# Autodesk Inventor assembly: Full_Model
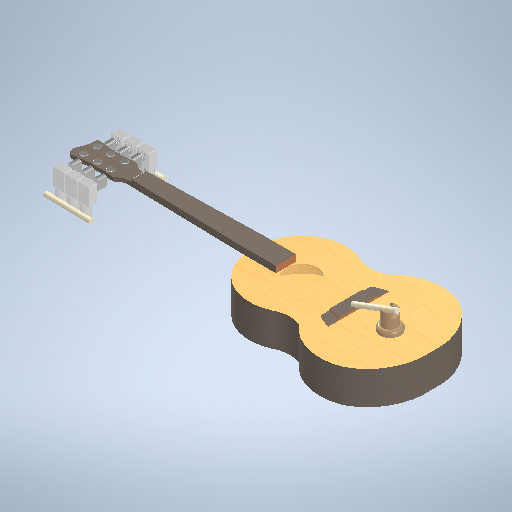
[picture p0: Inventor's stored thumbnail of the model, 512x512]
Saved by Autodesk Inventor 2025.2 (Build 292293000, 293)
## iProperties
Created: 2025-04-14
Part Number: Full_Model
Document SubType Name: Assembly
Designer: 3lin2
Author: 3lin2
## Documents named in this file (7)
- C:\Users\3lin2\OneDrive - University of Illinois - Urbana\Documents\UIUC\ECE 445\Automatic-Guitar-Tuner Github\3D_print\Full_Model.iam
- C:\Users\3lin2\OneDrive - University of Illinois - Urbana\Documents\UIUC\ECE 445\Automatic-Guitar-Tuner Github\3D_print\half_inch_dowel_5inch.ipt
- C:\Users\3lin2\OneDrive - University of Illinois - Urbana\Documents\UIUC\ECE 445\Automatic-Guitar-Tuner Github\3D_print\magnet_mount.ipt
- C:\Users\3lin2\OneDrive - University of Illinois - Urbana\Documents\UIUC\ECE 445\Automatic-Guitar-Tuner Github\3D_print\motor.ipt
- C:\Users\3lin2\OneDrive - University of Illinois - Urbana\Documents\UIUC\ECE 445\Automatic-Guitar-Tuner Github\3D_print\motor-tuningpeg.ipt
- C:\Users\3lin2\OneDrive - University of Illinois - Urbana\Documents\UIUC\ECE 445\Automatic-Guitar-Tuner Github\3D_print\Guitar.ipt
- C:\Users\3lin2\OneDrive - University of Illinois - Urbana\Documents\UIUC\ECE 445\Automatic-Guitar-Tuner Github\3D_print\tuningpeg.ipt
## Components (23 placed, 6 different names)
1. half_inch_dowel_5inch:1 — Angle:1, Mate:2
2. magnet_mount:1 — Angle:1, Mate:1, Mate:2
3. motor:1 — Rotational:7, Flush:1, Mate:3
4. motor-tuningpeg:1 — Rotational:7
5. Guitar:1 — Mate:1, Rotational:1, Rotational:2, Rotational:3, Rotational:4, Rotational:5, Rotational:6, Flush:1, Mate:3, Flush:2, Mate:4, Mate:5, Flush:3, Mate:6, Flush:4, Mate:7, Mate:8, Flush:5, Flush:6
6. tuningpeg:1 — Rotational:1
7. tuningpeg:2 — Rotational:2
8. tuningpeg:3 — Rotational:3
9. tuningpeg:4 — Rotational:6
10. tuningpeg:5 — Rotational:4
11. tuningpeg:6 — Rotational:5
12. motor:2 — Flush:2, Mate:4, Mate:10
13. motor-tuningpeg:2
14. motor:3 — Mate:5, Flush:3, Flush:7
15. motor-tuningpeg:3
16. motor:4 — Mate:6, Flush:4, Flush:8
17. motor-tuningpeg:4
18. motor:5 — Mate:8, Flush:6
19. motor-tuningpeg:5
20. motor:6 — Mate:7, Flush:5, Mate:9
21. motor-tuningpeg:6
22. half_inch_dowel_5inch:2 — Flush:7, Mate:10
23. half_inch_dowel_5inch:3 — Flush:8, Mate:9
## Relationships (31: RevoluteJoint 12, Mate 10, Flush 8, Angle 1)
- Angle:1 (-70 deg): half_inch_dowel_5inch:1 ↔ magnet_mount:1
- Mate:1: magnet_mount:1 ↔ Guitar:1
- Mate:2 (6.985 mm): half_inch_dowel_5inch:1 ↔ magnet_mount:1
- Rotational:1 [RevoluteJoint]: Guitar:1 ↔ tuningpeg:1
- Rotational:2 [RevoluteJoint]: Guitar:1 ↔ tuningpeg:2
- Rotational:3 [RevoluteJoint]: Guitar:1 ↔ tuningpeg:3
- Rotational:4 [RevoluteJoint]: Guitar:1 ↔ tuningpeg:5
- Rotational:5 [RevoluteJoint]: Guitar:1 ↔ tuningpeg:6
- Rotational:6 [RevoluteJoint]: Guitar:1 ↔ tuningpeg:4
- Rotational:7 [RevoluteJoint]: motor:1 ↔ motor-tuningpeg:1
- Flush:1 (-66.04 mm): motor:1 ↔ Guitar:1
- Mate:3 (50.8 mm): motor:1 ↔ Guitar:1
- [RevoluteJoint]: motor:2 ↔ motor-tuningpeg:2
- [RevoluteJoint]: motor:3 ↔ motor-tuningpeg:3
- Flush:2 (66.04 mm): Guitar:1 ↔ motor:2
- Mate:4 (50.8 mm): Guitar:1 ↔ motor:2
- Mate:5 (50.8 mm): Guitar:1 ↔ motor:3
- Flush:3 (66.04 mm): Guitar:1 ↔ motor:3
- [RevoluteJoint]: motor:4 ↔ motor-tuningpeg:4
- Mate:6 (50.8 mm): Guitar:1 ↔ motor:4
- Flush:4 (66.04 mm): Guitar:1 ↔ motor:4
- [RevoluteJoint]: motor:5 ↔ motor-tuningpeg:5
- [RevoluteJoint]: motor:6 ↔ motor-tuningpeg:6
- Mate:7 (50.8 mm): Guitar:1 ↔ motor:6
- Mate:8 (50.8 mm): Guitar:1 ↔ motor:5
- Flush:5 (66.04 mm): Guitar:1 ↔ motor:6
- Flush:6 (66.04 mm): Guitar:1 ↔ motor:5
- Flush:7 (-12.7 mm): motor:3 ↔ half_inch_dowel_5inch:2
- Flush:8 (12.7 mm): motor:4 ↔ half_inch_dowel_5inch:3
- Mate:9 (6.35 mm): motor:6 ↔ half_inch_dowel_5inch:3
- Mate:10 (6.35 mm): motor:2 ↔ half_inch_dowel_5inch:2
## Named parameters: d28_d23 = 0 mm, d29_d24 = -1.948927 deg, d30_d23 = 0 mm, d31_d24 = -1.910793 deg, d36_d23 = 0 mm, d37_d24 = -1.910793 deg, d40_d23 = 0 mm, d41_d24 = -1.910793 deg, d42_d23 = 0 mm, d43_d24 = -1.910793 deg
